# Autodesk Inventor assembly: 4DoF Manipulator Type 1
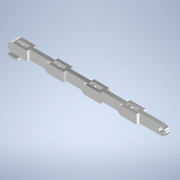
[picture p0: Inventor's stored thumbnail of the model, 180x180]
Saved by Autodesk Inventor 2021 (Build 250183000, 183)
## iProperties
Created: 2023-06-27
Part Number: 4DoF Manipulator Type 1
Document SubType Name: Assembly
Designer: fist5
Author: fist5
## Documents named in this file (3)
- C:\Users\fist5\Desktop\4DoF Manipulator Type 1.iam
- C:\Users\fist5\Desktop\Manipulator Base Type1.ipt
- C:\Users\fist5\Desktop\Manipulator Link Type 1.ipt
## Components (5 placed, 2 different names)
1. Manipulator Base Type1:2 — Mate:1, Mate:2
2. Manipulator Link Type 1:1 — Mate:1, Mate:2, Mate:3, Mate:4
3. Manipulator Link Type 1:2 — Mate:3, Mate:4, Mate:5, Mate:6
4. Manipulator Link Type 1:3 — Mate:5, Mate:6, Mate:7, Mate:8
5. Manipulator Link Type 1:4 — Mate:7, Mate:8
## Relationships (8: Mate 8)
- Mate:1: Manipulator Base Type1:2 ↔ Manipulator Link Type 1:1
- Mate:2: Manipulator Base Type1:2 ↔ Manipulator Link Type 1:1
- Mate:3: Manipulator Link Type 1:1 ↔ Manipulator Link Type 1:2
- Mate:4: Manipulator Link Type 1:1 ↔ Manipulator Link Type 1:2
- Mate:5: Manipulator Link Type 1:2 ↔ Manipulator Link Type 1:3
- Mate:6: Manipulator Link Type 1:2 ↔ Manipulator Link Type 1:3
- Mate:7: Manipulator Link Type 1:3 ↔ Manipulator Link Type 1:4
- Mate:8: Manipulator Link Type 1:3 ↔ Manipulator Link Type 1:4
